# Autodesk Inventor assembly: Assembly
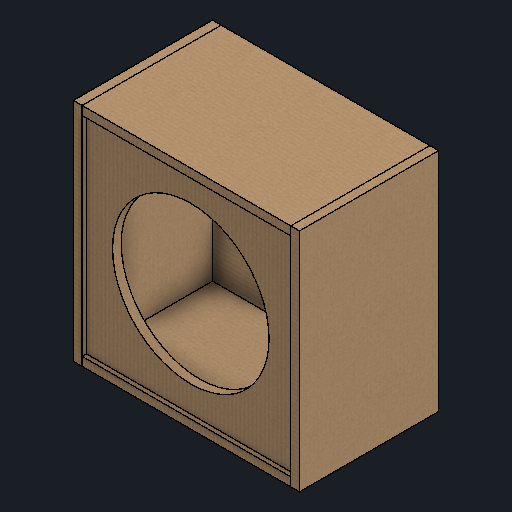
[picture p0: Inventor's stored thumbnail of the model, 512x512]
Saved by Autodesk Inventor 2026.2 (Build 302298000, 298)
## iProperties
Created: 2026-06-16
Part Number: Assembly
Document SubType Name: Assembly
Designer: JoshuaEah
Author: JoshuaEah
## Documents named in this file (6)
- C:\Users\JoshuaEah\Documents\GitHub\Designed-Trinkets\Guitar\110 Guitar Cab\Assembly.iam
- C:\Users\JoshuaEah\Documents\GitHub\Designed-Trinkets\Guitar\110 Guitar Cab\Part3.ipt
- C:\Users\JoshuaEah\Documents\GitHub\Designed-Trinkets\Guitar\110 Guitar Cab\Part2.ipt
- C:\Users\JoshuaEah\Documents\GitHub\Designed-Trinkets\Guitar\110 Guitar Cab\Part1.ipt
- C:\Users\JoshuaEah\Documents\GitHub\Designed-Trinkets\Guitar\110 Guitar Cab\Braces.ipt
- C:\Users\JoshuaEah\Documents\GitHub\Designed-Trinkets\Guitar\110 Guitar Cab\Back Plate.ipt
## Components (9 placed, 5 different names)
1. Part3:1 — Mate:1, Flush:1, Flush:2, Mate:2, Flush:3, Flush:4, Mate:7, Mate:9, Mate:14
2. Part2:1 — Mate:1, Flush:1, Flush:2, Flush:5, Flush:6, Mate:3, Mate:4, Flush:7, Mate:6, Mate:13
3. Part2:2 — Mate:2, Flush:3, Flush:4, Mate:11, Mate:15, Flush:9
4. Part3:2 — Flush:5, Flush:6, Mate:3, Mate:5, Mate:12, Flush:8
5. Part1:1 — Mate:4, Flush:7, Mate:5, Mate:8, Mate:10
6. Braces:1 — Mate:6, Mate:7, Mate:8
7. Braces:2 — Mate:9, Mate:10, Mate:11
8. Back Plate:1 — Mate:12, Flush:8, Mate:13
9. Back Plate:2 — Mate:14, Mate:15, Flush:9
## Relationships (24: Mate 15, Flush 9)
- Mate:1: Part3:1 ↔ Part2:1
- Flush:1: Part3:1 ↔ Part2:1
- Flush:2: Part3:1 ↔ Part2:1
- Mate:2: Part3:1 ↔ Part2:2
- Flush:3: Part3:1 ↔ Part2:2
- Flush:4: Part3:1 ↔ Part2:2
- Flush:5: Part2:1 ↔ Part3:2
- Flush:6: Part2:1 ↔ Part3:2
- Mate:3: Part2:1 ↔ Part3:2
- Mate:4: Part2:1 ↔ Part1:1
- Flush:7 (6.35 mm): Part2:1 ↔ Part1:1
- Mate:5: Part3:2 ↔ Part1:1
- Mate:6: Part2:1 ↔ Braces:1
- Mate:7: Part3:1 ↔ Braces:1
- Mate:8: Part1:1 ↔ Braces:1
- Mate:9: Part3:1 ↔ Braces:2
- Mate:10: Part1:1 ↔ Braces:2
- Mate:11: Part2:2 ↔ Braces:2
- Mate:12: Part3:2 ↔ Back Plate:1
- Flush:8: Part3:2 ↔ Back Plate:1
- Mate:13: Part2:1 ↔ Back Plate:1
- Mate:14: Part3:1 ↔ Back Plate:2
- Mate:15: Part2:2 ↔ Back Plate:2
- Flush:9: Part2:2 ↔ Back Plate:2
